# Autodesk Inventor assembly: lockingMechanismV02
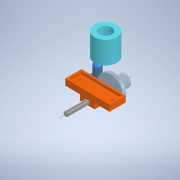
[picture p0: Inventor's stored thumbnail of the model, 180x180]
Saved by Autodesk Inventor 2021.1 (Build 251245010, 245A)
## iProperties
Created: 2020-08-16
Part Number: lockingMechanismV02
Document SubType Name: Assembly
Designer: robst
Author: robst
## Documents named in this file (6)
- C:\git\CAD-Development\robSteele\ShapeWays\TelescopeProjects\TelescopeMount\BobSteeleLockingMechanism\lockingMechanismV02.iam
- C:\git\CAD-Development\robSteele\ShapeWays\TelescopeProjects\TelescopeMount\BobSteeleLockingMechanism\outerShell.ipt
- C:\git\CAD-Development\robSteele\ShapeWays\TelescopeProjects\TelescopeMount\BobSteeleLockingMechanism\handle.ipt
- C:\git\CAD-Development\robSteele\ShapeWays\TelescopeProjects\TelescopeMount\ForkMountWithCelestronTubeConnector\Design Accelerator\Worm Gears2.iam
- C:\git\CAD-Development\robSteele\ShapeWays\TelescopeProjects\TelescopeMount\BobSteeleLockingMechanism\5_8_inSteelRod.ipt
- C:\git\CAD-Development\robSteele\ShapeWays\TelescopeProjects\TelescopeMount\connectorToTubeBrackets03.ipt
## Components (5 placed, 5 different names)
1. outerShell:1 — Insert:1
2. handle:1 — Insert:1
3. Worm Gears:1 [sub-assembly] — Insert:2
4. 5_8_inSteelRod:1 — Mate:1, Mate:2, Insert:2
5. connectorToTubeBrackets03:1 — Mate:1, Mate:2
## Relationships (4: Insert 2, Mate 2)
- Insert:1 (12.7 mm): outerShell:1 ↔ handle:1
- Mate:1: 5_8_inSteelRod:1 ↔ connectorToTubeBrackets03:1
- Mate:2: 5_8_inSteelRod:1 ↔ connectorToTubeBrackets03:1
- Insert:2: Worm Gears:1 ↔ 5_8_inSteelRod:1
